# Autodesk Inventor assembly: winch with ratchet prototype
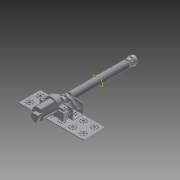
[picture p0: Inventor's stored thumbnail of the model, 180x180]
Saved by Autodesk Inventor 2013 (Build 170138000, 138)
## iProperties
Created: 2014-01-06
Part Number: winch with ratchet prototype
Document SubType Name: Assembly
Designer: kahohbein
Author: kahohbein
## Documents named in this file (7)
- C:\Users\kahohbein\Documents\GitHub\2013-2014_BlockParty\CAD\Lift\MK4\winch with ratchet prototype.iam
- C:\Users\kahohbein\Documents\GitHub\2013-2014_BlockParty\CAD\COTSParts\Tetrix\Tetrix flat plate.ipt
- C:\Users\kahohbein\Documents\GitHub\2013-2014_BlockParty\CAD\COTSParts\Fasteners\4-40 SHCS x125.ipt
- C:\Users\kahohbein\Documents\GitHub\2013-2014_BlockParty\CAD\COTSParts\Tetrix\Tetrix channel 32mm.ipt
- C:\Users\kahohbein\Documents\GitHub\2013-2014_BlockParty\CAD\Lift\MK4\Winch MK4.iam
- C:\Users\kahohbein\Documents\GitHub\2013-2014_BlockParty\CAD\COTSParts\Tetrix\Tetrix motor mount.ipt
- C:\Users\kahohbein\Documents\GitHub\2013-2014_BlockParty\CAD\Lift\MK4\ratchet stop mk 2.ipt
## Components (7 placed, 6 different names)
1. Tetrix flat plate:1 — Mate:1, Mate:2, Mate:3, Mate:5, Flush:2, Mate:6
2. 4-40 SHCS x125:1 — Mate:9, Mate:10
3. Tetrix channel 32mm:1 — Mate:5, Flush:2, Mate:6, Mate:7, Mate:8, Mate:9, Mate:10, Mate:11, Mate:12
4. Winch MK4:1 [sub-assembly] — Mate:4, Flush:1
5. Tetrix motor mount:1 — Mate:1, Mate:2, Mate:3, Mate:4, Flush:1
6. ratchet stop mk 2:1 — Mate:7, Mate:8
7. 4-40 SHCS x125:2 — Mate:11, Mate:12
## Relationships (14: Mate 12, Flush 2)
- Mate:1: Tetrix flat plate:1 ↔ Tetrix motor mount:1
- Mate:2: Tetrix flat plate:1 ↔ Tetrix motor mount:1
- Mate:3: Tetrix flat plate:1 ↔ Tetrix motor mount:1
- Mate:4: Winch MK4:1 ↔ Tetrix motor mount:1
- Flush:1 (-9.652 mm): Winch MK4:1 ↔ Tetrix motor mount:1
- Mate:5: Tetrix flat plate:1 ↔ Tetrix channel 32mm:1
- Flush:2: Tetrix flat plate:1 ↔ Tetrix channel 32mm:1
- Mate:6: Tetrix flat plate:1 ↔ Tetrix channel 32mm:1
- Mate:7: Tetrix channel 32mm:1 ↔ ratchet stop mk 2:1
- Mate:8: Tetrix channel 32mm:1 ↔ ratchet stop mk 2:1
- Mate:9: 4-40 SHCS x125:1 ↔ Tetrix channel 32mm:1
- Mate:10: 4-40 SHCS x125:1 ↔ Tetrix channel 32mm:1
- Mate:11: Tetrix channel 32mm:1 ↔ 4-40 SHCS x125:2
- Mate:12: Tetrix channel 32mm:1 ↔ 4-40 SHCS x125:2
